# Autodesk Inventor assembly: MIRright脚一枚
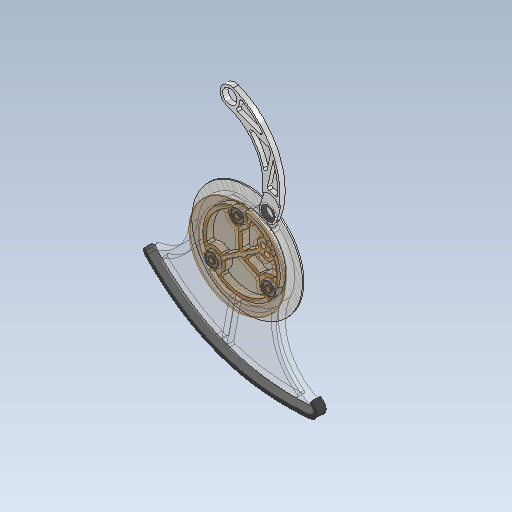
[picture p0: Inventor's stored thumbnail of the model, 512x512]
Saved by Autodesk Inventor 2020.2 (Build 242310000, 310)
## iProperties
Created: 2020-04-13
Part Number: MIRright脚一枚
Document SubType Name: Assembly
Designer: aoyama
Mass: 31.6013 g
Surface Area: 259.988 cm^2
Volume: 17.8864 cm^3
Density: 1.76678 g/cm^3
Author: aoyama
## Documents named in this file (8)
- C:\Users\aoyam\Desktop\SRDC_local\Inventor\二年機\Geminiβ\脚\ネジクランク\MIR達\MIRright脚一枚.iam
- C:\Users\aoyam\Desktop\SRDC_local\Inventor\二年機\Geminiβ\脚\ネジクランク\MIR達\MIRrightクランク3t.ipt
- C:\Users\aoyam\Desktop\SRDC_local\Inventor\二年機\Geminiβ\脚\ネジクランク\MIR達\MIRrightクランク4t.ipt
- C:\Users\aoyam\Desktop\SRDC_local\Inventor\二年機\Geminiβ\汎用部品\MIR達\MIRrightベアリングd3D8B4F無.ipt
- C:\Users\aoyam\Desktop\SRDC_local\Inventor\二年機\Geminiβ\脚\ネジクランク\MIR達\MIRrightヘッケン改.ipt
- C:\Users\aoyam\Desktop\SRDC_local\Inventor\二年機\Geminiβ\脚\ネジクランク\MIR達\MIRright揺動節.ipt
- C:\Users\aoyam\Desktop\SRDC_local\Inventor\二年機\Geminiβ\汎用部品\MIR達\MIRrightオイレス外径8内径6L2.ipt
- C:\Users\aoyam\Desktop\SRDC_local\Inventor\二年機\Geminiβ\脚\ネジクランク\MIR達\MIRright脚ゴム.ipt
## Components (9 placed, 7 different names)
1. MIRrightクランク3t:1 — 挿入:15, 挿入:11
2. MIRrightクランク4t:1 — 挿入:8, 挿入:9, 挿入:10, 挿入:11, 挿入:14
3. MIRrightベアリングd3D8B4F無:1 — 挿入:8
4. MIRrightベアリングd3D8B4F無:2 — 挿入:15, 挿入:10
5. MIRrightベアリングd3D8B4F無:3 — 挿入:9
6. MIRrightヘッケン改:1 — 挿入:11, 挿入:12, 挿入:13, 挿入:14
7. MIRright揺動節:1 — 挿入:11, 挿入:15
8. MIRrightオイレス外径8内径6L2:1 — 挿入:15
9. MIRright脚ゴム:1 — 挿入:12, 挿入:13
## Relationships (10: Insert 10)
- 挿入:15 [Insert]: MIRrightクランク3t:1 ↔ MIRrightベアリングd3D8B4F無:2
- 挿入:11 [Insert]: MIRrightヘッケン改:1 ↔ MIRright揺動節:1
- 挿入:8 [Insert]: MIRrightクランク4t:1 ↔ MIRrightベアリングd3D8B4F無:1
- 挿入:9 [Insert]: MIRrightクランク4t:1 ↔ MIRrightベアリングd3D8B4F無:3
- 挿入:10 [Insert]: MIRrightクランク4t:1 ↔ MIRrightベアリングd3D8B4F無:2
- 挿入:11 [Insert]: MIRrightクランク3t:1 ↔ MIRrightクランク4t:1
- 挿入:12 [Insert]: MIRrightヘッケン改:1 ↔ MIRright脚ゴム:1
- 挿入:13 [Insert]: MIRrightヘッケン改:1 ↔ MIRright脚ゴム:1
- 挿入:14 [Insert] (0.2 mm): MIRrightクランク4t:1 ↔ MIRrightヘッケン改:1
- 挿入:15 [Insert]: MIRright揺動節:1 ↔ MIRrightオイレス外径8内径6L2:1
